# Autodesk Inventor assembly: Shooter
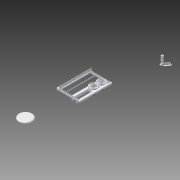
[picture p0: Inventor's stored thumbnail of the model, 180x180]
Saved by Autodesk Inventor 2013 (Build 170138000, 138)
## iProperties
Created: 2013-01-27
Part Number: Shooter
Document SubType Name: Assembly
Designer: Naphat
Author: Naphat
## Documents named in this file (14)
- C:\Users\carneeki\Desktop\Kiwi Robot\Shooter\Shooter.iam
- C:\Users\carneeki\Desktop\Kiwi Robot\Imported Components\Wheels\Basic Wheel\Shooter Basic Design.iam
- C:\Users\carneeki\Desktop\Kiwi Robot\Shooter\26in Angle Channel.ipt
- C:\Users\carneeki\Desktop\Kiwi Robot\Shooter\26in mini C-Channel (rail).ipt
- C:\Users\carneeki\Desktop\Kiwi Robot\Shooter\18in C-Channel Front.ipt
- C:\Users\carneeki\Desktop\Kiwi Robot\Shooter\18in C-Channel Rear.ipt
- C:\Users\carneeki\Desktop\Kiwi Robot\Shooter\26in Angle Channel CIM Mount Left.ipt
- C:\Users\carneeki\Desktop\Kiwi Robot\Shooter\26in Angle Channel CIM Mount Right.ipt
- C:\Users\carneeki\Desktop\Kiwi Robot\Shooter\26in C-Channel Left.ipt
- C:\Users\carneeki\Desktop\Kiwi Robot\Shooter\26in C-Channel Right.ipt
- C:\Users\carneeki\Desktop\Kiwi Robot\Imported Components\Motors\CIM Mount\CIM Mount Bolt.ipt
- C:\Users\carneeki\Desktop\Kiwi Robot\Shooter\Firing Pin\Firing Pin.iam
- C:\Users\carneeki\Desktop\Kiwi Robot\Shooter\Frisbee.ipt
- C:\Users\carneeki\Desktop\Kiwi Robot\Imported Components\Motors\PG27\PG27.ipt
## Components (18 placed, 14 different names)
1. 26in C-Channel Right:1 — Insert:22, Flush:5, Insert:23, Flush:6
2. 18in C-Channel Rear — Mate:213, Insert:13, Insert:14, Insert:20, Mate:216, Flush:1, Flush:4, Insert:23, Flush:6, Mate:218, Flush:7, Mate:220, Flush:8
3. 18in C-Channel Front — Mate:212, Mate:215, Insert:21, Flush:3, Insert:22, Flush:5, Mate:219, Mate:221
4. 26in C-Channel Left:1 — Insert:20, Mate:217, Flush:2, Insert:21, Flush:3, Flush:4
5. 26in Angle Channel:1 — Mate:217, Flush:2
6. 26in Angle Channel CIM Mount Right:1 — Mate:212, Mate:213, Insert:13, Insert:14, Mate:223
7. 26in Angle Channel CIM Mount Left:3 — Mate:214, Mate:215, Mate:216, Flush:1, Insert:29, Insert:30, Insert:31, Insert:32, Insert:33, Insert:34, Insert:35, Insert:36
8. 26in mini C-Channel (rail):1 — Mate:218, Mate:219, Flush:7
9. 26in mini C-Channel (rail):2 — Mate:220, Mate:221, Flush:8, Mate:222
10. CIM Mount Bolt:1 — Insert:31
11. CIM Mount Bolt:2 — Insert:32
12. CIM Mount Bolt:3 — Insert:34
13. CIM Mount Bolt:4 — Insert:33
14. Firing Pin:1 [sub-assembly] — Mate:210, Mate:211
15. Frisbee:1 — Mate:222
16. PG27:1 — Mate:210, Mate:211
17. Wheel Assy:Rear [sub-assembly] — Mate:214, Insert:35, Insert:36
18. Wheel Assy:Front [sub-assembly] — Insert:29, Insert:30, Mate:223
## Relationships (36: Mate 14, Insert 14, Flush 8)
- Mate:210: Firing Pin:1 ↔ PG27:1
- Mate:211: Firing Pin:1 ↔ PG27:1
- Mate:212: 18in C-Channel Front ↔ 26in Angle Channel CIM Mount Right:1
- Mate:213: 18in C-Channel Rear ↔ 26in Angle Channel CIM Mount Right:1
- Insert:13: 18in C-Channel Rear ↔ 26in Angle Channel CIM Mount Right:1
- Insert:14: 18in C-Channel Rear ↔ 26in Angle Channel CIM Mount Right:1
- Insert:20: 18in C-Channel Rear ↔ 26in C-Channel Left:1
- Mate:214: 26in Angle Channel CIM Mount Left:3 ↔ Wheel Assy:Rear
- Mate:215: 18in C-Channel Front ↔ 26in Angle Channel CIM Mount Left:3
- Mate:216: 18in C-Channel Rear ↔ 26in Angle Channel CIM Mount Left:3
- Flush:1: 18in C-Channel Rear ↔ 26in Angle Channel CIM Mount Left:3
- Mate:217: 26in C-Channel Left:1 ↔ 26in Angle Channel:1
- Flush:2: 26in C-Channel Left:1 ↔ 26in Angle Channel:1
- Insert:21: 18in C-Channel Front ↔ 26in C-Channel Left:1
- Flush:3: 18in C-Channel Front ↔ 26in C-Channel Left:1
- Flush:4: 18in C-Channel Rear ↔ 26in C-Channel Left:1
- Insert:22: 26in C-Channel Right:1 ↔ 18in C-Channel Front
- Flush:5: 26in C-Channel Right:1 ↔ 18in C-Channel Front
- Insert:23: 26in C-Channel Right:1 ↔ 18in C-Channel Rear
- Flush:6: 26in C-Channel Right:1 ↔ 18in C-Channel Rear
- Mate:218: 18in C-Channel Rear ↔ 26in mini C-Channel (rail):1
- Mate:219: 18in C-Channel Front ↔ 26in mini C-Channel (rail):1
- Flush:7: 18in C-Channel Rear ↔ 26in mini C-Channel (rail):1
- Mate:220: 18in C-Channel Rear ↔ 26in mini C-Channel (rail):2
- Mate:221: 18in C-Channel Front ↔ 26in mini C-Channel (rail):2
- Flush:8: 18in C-Channel Rear ↔ 26in mini C-Channel (rail):2
- Mate:222: 26in mini C-Channel (rail):2 ↔ Frisbee:1
- Insert:29: 26in Angle Channel CIM Mount Left:3 ↔ Wheel Assy:Front
- Insert:30: 26in Angle Channel CIM Mount Left:3 ↔ Wheel Assy:Front
- Insert:31: 26in Angle Channel CIM Mount Left:3 ↔ CIM Mount Bolt:1
- Insert:32: 26in Angle Channel CIM Mount Left:3 ↔ CIM Mount Bolt:2
- Insert:33: 26in Angle Channel CIM Mount Left:3 ↔ CIM Mount Bolt:4
- Insert:34: 26in Angle Channel CIM Mount Left:3 ↔ CIM Mount Bolt:3
- Insert:35: 26in Angle Channel CIM Mount Left:3 ↔ Wheel Assy:Rear
- Insert:36: 26in Angle Channel CIM Mount Left:3 ↔ Wheel Assy:Rear
- Mate:223: 26in Angle Channel CIM Mount Right:1 ↔ Wheel Assy:Front
